# Autodesk Inventor assembly: lanceur
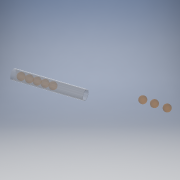
[picture p0: Inventor's stored thumbnail of the model, 180x180]
Saved by Autodesk Inventor 2017 (Build 210142000, 142)
## iProperties
Created: 2018-01-27
Part Number: lanceur
Document SubType Name: Assembly
Designer: franc
Author: franc
## Documents named in this file (3)
- C:\Users\franc\Desktop\EsialRobotik\Mecanique\2018\robot\traitement-eau\lanceur.iam
- C:\Users\franc\Desktop\EsialRobotik\Mecanique\2018\robot\traitement-eau\cylindre-lanceur.ipt
- C:\Users\franc\Desktop\EsialRobotik\Mecanique\2018\robot\traitement-eau\eau.ipt
## Components (9 placed, 2 different names)
1. cylindre-lanceur:1 — Placage:1, Placage:2, Placage:3, Placage:4, Placage:5
2. eau:1 — Placage:1
3. eau:2 — Placage:2
4. eau:3 — Placage:3
5. eau:4 — Placage:5
6. eau:5 — Placage:4
7. eau:6
8. eau:7
9. eau:8
## Relationships (5: Mate 5)
- Placage:1 [Mate]: cylindre-lanceur:1 ↔ eau:1
- Placage:2 [Mate]: cylindre-lanceur:1 ↔ eau:2
- Placage:3 [Mate]: cylindre-lanceur:1 ↔ eau:3
- Placage:4 [Mate]: cylindre-lanceur:1 ↔ eau:5
- Placage:5 [Mate]: cylindre-lanceur:1 ↔ eau:4
